# Autodesk Inventor assembly: Assembly wit no emboss on nozzle
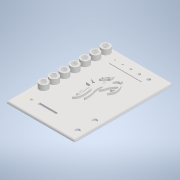
[picture p0: Inventor's stored thumbnail of the model, 180x180]
Saved by Autodesk Inventor 2020.2 (Build 242310000, 310)
## iProperties
Created: 2020-05-06
Part Number: Assembly wit no emboss on nozzle
Document SubType Name: Assembly
Designer: Amaan Khalid
Author: Amaan Khalid
## Documents named in this file (3)
- C:\Users\Amaan Khalid\Desktop\My projects\Tool Holder (Done)\Assembly wit no emboss on nozzle.iam
- C:\Users\Amaan Khalid\Desktop\tool holder\proto.ipt
- C:\Users\Amaan Khalid\Desktop\tool holder\yeyeyey update'.ipt
## Components (8 placed, 2 different names)
1. proto:1 — Mate:2, Mate:3, Mate:4, Mate:5, Mate:6, Mate:7, Mate:8
2. yeyeyey update':1 — Mate:8
3. yeyeyey update':2 — Mate:2
4. yeyeyey update':3 — Mate:3
5. yeyeyey update':4 — Mate:4
6. yeyeyey update':6 — Mate:5
7. yeyeyey update':8 — Mate:6
8. yeyeyey update':9 — Mate:7
## Relationships (7: Mate 7)
- Mate:2: proto:1 ↔ yeyeyey update':2
- Mate:3: proto:1 ↔ yeyeyey update':3
- Mate:4: proto:1 ↔ yeyeyey update':4
- Mate:5: proto:1 ↔ yeyeyey update':6
- Mate:6: proto:1 ↔ yeyeyey update':8
- Mate:7: proto:1 ↔ yeyeyey update':9
- Mate:8: proto:1 ↔ yeyeyey update':1
